# Autodesk Inventor assembly: omni wheel holder assembly
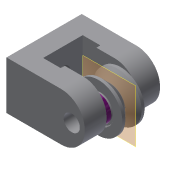
[picture p0: Inventor's stored thumbnail of the model, 180x180]
Saved by Autodesk Inventor 2018 (Build 220112000, 112)
## iProperties
Created: 2019-01-03
Part Number: omni wheel holder assembly
Document SubType Name: Assembly
Designer: ball
Author: ball
## Documents named in this file (5)
- C:\FTC\FTC8863CAD\2018Robot\omni wheel holder assembly.iam
- C:\FTC\FTC8863CAD\GoBilda\1609 Parts\1609-0613-0004.ipt
- C:\FTC\FTC8863CAD\GoBilda\2807 Parts\2807-0407-1000.ipt
- C:\FTC\FTC8863CAD\2018Robot\omni wheel holder proto.ipt
- C:\FTC\FTC8863CAD\2018Robot\omni wheel wheel holder proto.ipt
## Components (5 placed, 4 different names)
1. 1609-0613-0004:1 — Mate:1, Mate:2, Mate:3, Mate:4, Mate:6
2. 2807-0407-1000:1 — Mate:1, Mate:2, Mate:5
3. 2807-0407-1000:2 — Mate:3, Mate:4
4. omni wheel holder proto:1
5. omni wheel wheel holder proto:2 — Mate:5, Mate:6
## Relationships (6: Mate 6)
- Mate:1: 1609-0613-0004:1 ↔ 2807-0407-1000:1
- Mate:2: 1609-0613-0004:1 ↔ 2807-0407-1000:1
- Mate:3: 1609-0613-0004:1 ↔ 2807-0407-1000:2
- Mate:4: 1609-0613-0004:1 ↔ 2807-0407-1000:2
- Mate:5 (0.254 mm): 2807-0407-1000:1 ↔ omni wheel wheel holder proto:2
- Mate:6: 1609-0613-0004:1 ↔ omni wheel wheel holder proto:2
